# Autodesk Inventor assembly: Coffee Maker
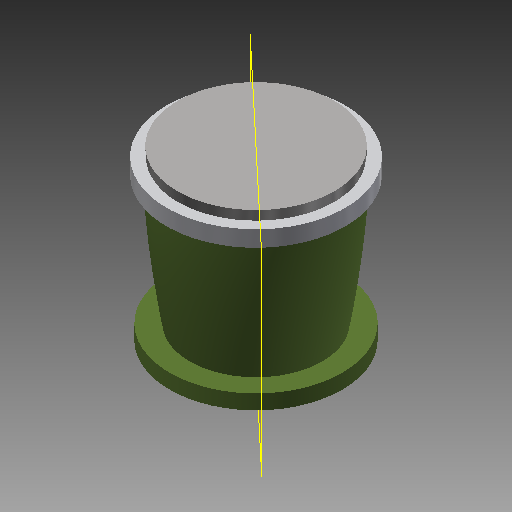
[picture p0: Inventor's stored thumbnail of the model, 512x512]
Saved by Autodesk Inventor 2018 (Build 220112000, 112)
## iProperties
Created: 2017-10-26
Part Number: Coffee Maker
Document SubType Name: Assembly
Designer: kurtis
Author: kurtis
## Documents named in this file (4)
- D:\Users\kurti\Git-Home\CAD\GE101\MA7\Coffee Maker.iam
- D:\Users\kurti\Git-Home\CAD\GE101\MA7\Cup.ipt
- D:\Users\kurti\Git-Home\CAD\GE101\MA7\Bucket.ipt
- D:\Users\kurti\Git-Home\CAD\GE101\MA7\lid.ipt
## Components (3 placed, 3 different names)
1. Cup:1 — Cylindrical:1, Mate:1
2. Bucket:1 — Cylindrical:1, Mate:1, Mate:2, Rotational:1
3. lid:1 — Mate:2, Rotational:1
## Relationships (4: Mate 2, CylindricalJoint 1, RevoluteJoint 1)
- Cylindrical:1: Cup:1 ↔ Bucket:1
- Mate:1: Cup:1 ↔ Bucket:1
- Mate:2: Bucket:1 ↔ lid:1
- Rotational:1 [RevoluteJoint]: Bucket:1 ↔ lid:1
